# Autodesk Inventor assembly: Assembly1
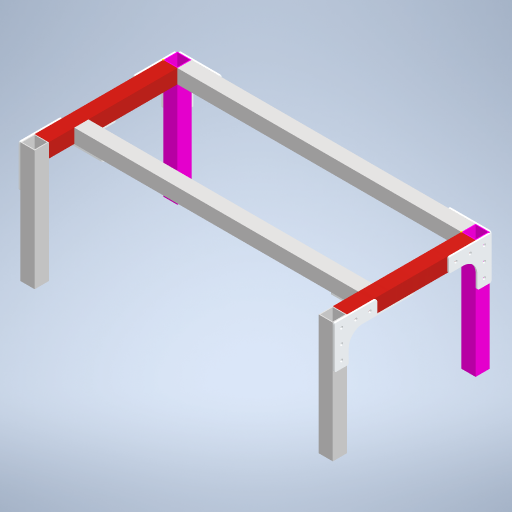
[picture p0: Inventor's stored thumbnail of the model, 512x512]
Saved by Autodesk Inventor 2024 (Build 280153000, 153)
## iProperties
Created: 2024-01-18
Part Number: Assembly1
Document SubType Name: Assembly
Designer: mongd
Author: mongd
## Documents named in this file (6)
- C:\Users\mongd\OneDrive\Documents\GitHub\BehrendURCMechanical\CAD\Controls\Chassis_Super_Structure\Assembly1.iam
- C:\Users\mongd\OneDrive\Documents\GitHub\BehrendURCMechanical\CAD\Controls\Chassis_Super_Structure\Pillar_Long.ipt
- C:\Users\mongd\OneDrive\Documents\GitHub\BehrendURCMechanical\CAD\Controls\Chassis_Super_Structure\Pillar_Short.ipt
- C:\Users\mongd\OneDrive\Documents\GitHub\BehrendURCMechanical\CAD\Controls\Chassis_Super_Structure\Horizontal_Beam_Long.ipt
- C:\Users\mongd\OneDrive\Documents\GitHub\BehrendURCMechanical\CAD\Controls\Chassis_Super_Structure\HOrizontal_Beam_Short.ipt
- C:\Users\mongd\OneDrive\Documents\GitHub\BehrendURCMechanical\CAD\Controls\Chassis_Super_Structure\am-3860 90 Gusset REV2\am-3860 90 Gusset REV2.ipt
## Components (16 placed, 5 different names)
1. Pillar_Long:1 — Mate:1, Mate:4, Flush:5, Flush:6, Flush:29
2. Pillar_Long:2 — Mate:5, Flush:7, Flush:8, Flush:9, Flush:24
3. Pillar_Short:1 — Mate:6, Flush:10, Flush:11, Flush:12, Mate:8, Flush:16, Flush:17, Flush:27, Mate:17, Flush:32
4. Pillar_Short:2 — Mate:7, Flush:13, Flush:14, Flush:15, Flush:18, Flush:19, Mate:11, Flush:22, Mate:14, Flush:25
5. Horizontal_Beam_Long:2 — Mate:8, Flush:16, Flush:17, Flush:18, Flush:19, Mate:10, Mate:11, Flush:26, Flush:31
6. HOrizontal_Beam_Short:1 — Mate:4, Flush:5, Flush:6, Mate:6, Flush:10, Flush:11, Flush:12, Flush:20, Mate:9, Mate:15, Flush:28, Mate:16, Flush:30, Mate:19, Flush:35
7. HOrizontal_Beam_Short:2 — Mate:5, Flush:7, Flush:8, Flush:9, Mate:7, Flush:13, Flush:14, Flush:15, Mate:12, Flush:21, Mate:13, Flush:23, Flush:33
8. Horizontal_Beam_Long:3 — Flush:20, Mate:9, Mate:10, Mate:18, Flush:34, Flush:36
9. am-3860 90 Gusset REV2:1 — Mate:13, Flush:23, Flush:24
10. am-3860 90 Gusset REV2:2 — Mate:12, Flush:21, Flush:22
11. am-3860 90 Gusset REV2:3 — Mate:17, Flush:31, Flush:32
12. am-3860 90 Gusset REV2:4 — Mate:15, Flush:27, Flush:28
13. am-3860 90 Gusset REV2:5 — Mate:14, Flush:25, Flush:26
14. am-3860 90 Gusset REV2:6 — Mate:16, Flush:29, Flush:30
15. am-3860 90 Gusset REV2:7 — Mate:18, Flush:33, Flush:34
16. am-3860 90 Gusset REV2:8 — Mate:19, Flush:35, Flush:36
## Relationships (49: Flush 32, Mate 17)
- Mate:1: Pillar_Long:1
- Mate:4: Pillar_Long:1 ↔ HOrizontal_Beam_Short:1
- Flush:5: Pillar_Long:1 ↔ HOrizontal_Beam_Short:1
- Flush:6: Pillar_Long:1 ↔ HOrizontal_Beam_Short:1
- Mate:5: Pillar_Long:2 ↔ HOrizontal_Beam_Short:2
- Flush:7: Pillar_Long:2 ↔ HOrizontal_Beam_Short:2
- Flush:8: Pillar_Long:2 ↔ HOrizontal_Beam_Short:2
- Flush:9: Pillar_Long:2 ↔ HOrizontal_Beam_Short:2
- Mate:6: Pillar_Short:1 ↔ HOrizontal_Beam_Short:1
- Flush:10: Pillar_Short:1 ↔ HOrizontal_Beam_Short:1
- Flush:11: Pillar_Short:1 ↔ HOrizontal_Beam_Short:1
- Flush:12: Pillar_Short:1 ↔ HOrizontal_Beam_Short:1
- Mate:7: Pillar_Short:2 ↔ HOrizontal_Beam_Short:2
- Flush:13: Pillar_Short:2 ↔ HOrizontal_Beam_Short:2
- Flush:14: Pillar_Short:2 ↔ HOrizontal_Beam_Short:2
- Flush:15: Pillar_Short:2 ↔ HOrizontal_Beam_Short:2
- Mate:8: Pillar_Short:1 ↔ Horizontal_Beam_Long:2
- Flush:16: Pillar_Short:1 ↔ Horizontal_Beam_Long:2
- Flush:17: Pillar_Short:1 ↔ Horizontal_Beam_Long:2
- Flush:18: Pillar_Short:2 ↔ Horizontal_Beam_Long:2
- Flush:19: Pillar_Short:2 ↔ Horizontal_Beam_Long:2
- Flush:20: HOrizontal_Beam_Short:1 ↔ Horizontal_Beam_Long:3
- Mate:9: HOrizontal_Beam_Short:1 ↔ Horizontal_Beam_Long:3
- Mate:10 (159.1818 mm): Horizontal_Beam_Long:2 ↔ Horizontal_Beam_Long:3
- Mate:11: Pillar_Short:2 ↔ Horizontal_Beam_Long:2
- Mate:12: HOrizontal_Beam_Short:2 ↔ am-3860 90 Gusset REV2:2
- Flush:21: HOrizontal_Beam_Short:2 ↔ am-3860 90 Gusset REV2:2
- Flush:22: Pillar_Short:2 ↔ am-3860 90 Gusset REV2:2
- Mate:13: HOrizontal_Beam_Short:2 ↔ am-3860 90 Gusset REV2:1
- Flush:23: HOrizontal_Beam_Short:2 ↔ am-3860 90 Gusset REV2:1
- Flush:24: Pillar_Long:2 ↔ am-3860 90 Gusset REV2:1
- Mate:14: Pillar_Short:2 ↔ am-3860 90 Gusset REV2:5
- Flush:25: Pillar_Short:2 ↔ am-3860 90 Gusset REV2:5
- Flush:26: Horizontal_Beam_Long:2 ↔ am-3860 90 Gusset REV2:5
- Mate:15: HOrizontal_Beam_Short:1 ↔ am-3860 90 Gusset REV2:4
- Flush:27: Pillar_Short:1 ↔ am-3860 90 Gusset REV2:4
- Flush:28: HOrizontal_Beam_Short:1 ↔ am-3860 90 Gusset REV2:4
- Mate:16: HOrizontal_Beam_Short:1 ↔ am-3860 90 Gusset REV2:6
- Flush:29: Pillar_Long:1 ↔ am-3860 90 Gusset REV2:6
- Flush:30: HOrizontal_Beam_Short:1 ↔ am-3860 90 Gusset REV2:6
- Mate:17: Pillar_Short:1 ↔ am-3860 90 Gusset REV2:3
- Flush:31: Horizontal_Beam_Long:2 ↔ am-3860 90 Gusset REV2:3
- Flush:32: Pillar_Short:1 ↔ am-3860 90 Gusset REV2:3
- Mate:18: Horizontal_Beam_Long:3 ↔ am-3860 90 Gusset REV2:7
- Flush:33: HOrizontal_Beam_Short:2 ↔ am-3860 90 Gusset REV2:7
- Flush:34: Horizontal_Beam_Long:3 ↔ am-3860 90 Gusset REV2:7
- Mate:19: HOrizontal_Beam_Short:1 ↔ am-3860 90 Gusset REV2:8
- Flush:35: HOrizontal_Beam_Short:1 ↔ am-3860 90 Gusset REV2:8
- Flush:36: Horizontal_Beam_Long:3 ↔ am-3860 90 Gusset REV2:8
